# Autodesk Inventor assembly: Cube 1x1 V5 (Mirror Horizontal)
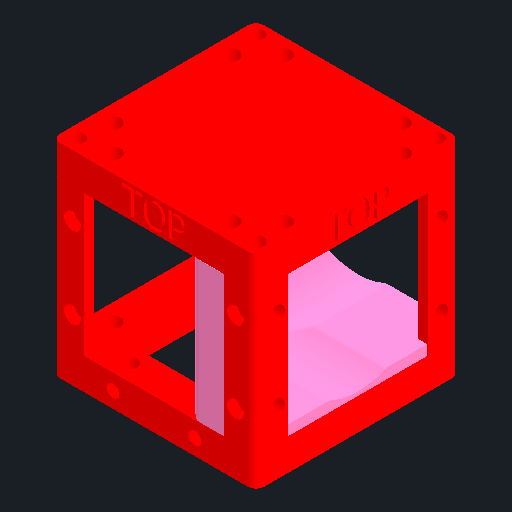
[picture p0: Inventor's stored thumbnail of the model, 512x512]
Saved by Autodesk Inventor 2023.4 (Build 274418000, 418)
## iProperties
Created: 2022-08-13
Part Number: Cube 1x1 V5 (Mirror Horizontal)
Document SubType Name: Assembly
Designer: xSibe
Author: xSibe
## Documents named in this file (4)
- C:\.Laptop\.Work\Projects\Project Protocube\Protocube\CAD, STL, OBJ Files\1 CAD\Mirror\Cube 1x1 V5 (Mirror Horizontal).iam
- C:\.Laptop\.Work\Projects\Project Protocube\Protocube\CAD, STL, OBJ Files\1 CAD\Mirror\Mirror Base Horizontal.ipt
- C:\.Laptop\.Work\Projects\Project Protocube\Protocube\CAD, STL, OBJ Files\1 CAD\Mirror\Mirror Plate Horizontal.ipt
- C:\.Laptop\.Work\Projects\Project Protocube\Protocube\CAD, STL, OBJ Files\1 CAD\Cubes\Cube 1x1 V5 Mirror.iam
## Components (3 placed, 3 different names)
1. Mirror Base Horizontal:1 — Flush:1, Flush:2, Mate:4, Flush:3
2. Mirror Plate Horizontal:1 — Flush:2, Mate:5, Flush:3
3. Cube 1x1 V5 Mirror:1 [sub-assembly]
## Relationships (5: Flush 3, Mate 2)
- Flush:1: Mirror Base Horizontal:1
- Flush:2: Mirror Base Horizontal:1 ↔ Mirror Plate Horizontal:1
- Mate:4: Mirror Base Horizontal:1
- Mate:5: Mirror Plate Horizontal:1
- Flush:3: Mirror Base Horizontal:1 ↔ Mirror Plate Horizontal:1
